# Autodesk Inventor assembly: Rover
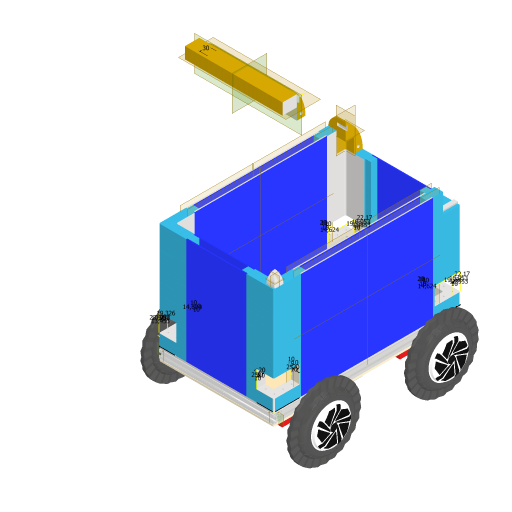
[picture p0: Inventor's stored thumbnail of the model, 512x512]
Saved by Autodesk Inventor 2023.2 (Build 272271030, 271C)
## iProperties
Created: 2024-10-30
Part Number: Rover
Document SubType Name: Assembly
Designer: I9232
Author: I9232
## Documents named in this file (21)
- D:\!Rover\Rover\Rover_construction\Rover.iam
- D:\!Rover\Rover\Rover_construction\platform.ipt
- D:\!Rover\Rover\Rover_construction\Motor, BLDC, Hoverboard Wheel, 8.0in.ipt
- D:\!Rover\Rover\Rover_construction\Profil 20x20.ipt
- D:\!Rover\Rover\Rover_construction\Крепление мотора.iam
- D:\!Rover\Rover\Rover_construction\Copter.ipt
- D:\!Rover\Rover\Rover_construction\Korpus.ipt
- D:\!Rover\Rover\Rover_construction\Уголок для профиля.ipt
- D:\!Rover\Rover\Rover_construction\Профиль 30x30\Профиль 30x30.ipt
- D:\!Rover\Rover\Rover_construction\Т-образный соединитель\Т-образный соединитель.ipt
- D:\!Rover\Rover\Rover_construction\KRAVT_holder_2 (1) (2).ipt
- D:\!Rover\Rover\Rover_construction\столик.ipt
- D:\!Rover\Rover\Rover_construction\Подъёмник.iam
- D:\!Rover\Rover\Rover_construction\Столбик.ipt
- D:\!Rover\Rover\Rover_construction\Боковая часть корпуса.ipt
- D:\!Rover\Rover\Rover_construction\Край задней части корпуса.ipt
- D:\!Rover\Rover\Rover_construction\кубик.ipt
- D:\!Rover\Rover\Rover_construction\Передняя_Задняя фанера.ipt
- D:\!Rover\Rover\Rover_construction\Проставка для боковых фанер.ipt
- D:\!Rover\Rover\Rover_construction\Крышка.ipt
- D:\!Rover\Rover\Rover_construction\Уголок крышки.ipt
## Components (48 placed, 21 different names)
1. platform:1 — Совмещение:1, Совмещение:2, Совмещение:169, Заподлицо:1, Заподлицо:2, Совмещение:170, Совмещение:171, Совмещение:172, Заподлицо:3, Заподлицо:4, Заподлицо:5, Заподлицо:6, Совмещение:180, Заподлицо:11, Совмещение:189, Заподлицо:24, Заподлицо:25, Совмещение:190, Заподлицо:26, Заподлицо:27, Заподлицо:28, Совмещение:191, Заподлицо:29, Совмещение:192, Заподлицо:30, Заподлицо:31, Совмещение:205, Совмещение:206, Заподлицо:33, Заподлицо:34, Заподлицо:37
2. Copter:1 — Совмещение:213, Совмещение:214
3. Корпус:1 — Совмещение:210, Совмещение:211, Заподлицо:33, Заподлицо:34, Совмещение:212
4. Т-образный соединитель:1 — Заподлицо:21, Совмещение:186, Совмещение:188
5. Т-образный соединитель:2 — Заподлицо:22, Совмещение:187, Заподлицо:23
6. KRAVT_holder_2 (1) (2):1 — Совмещение:206, Заподлицо:32, Совмещение:209
7. KRAVT_holder_2 (1) (2):2 — Совмещение:205, Совмещение:207, Совмещение:208
8. столик:1 — Совмещение:210, Совмещение:211, Совмещение:213
9. Copter:2 — Совмещение:214
10. Подъёмник:1 [sub-assembly]
11. platform:2 — Совмещение:221, Заподлицо:37, Заподлицо:38, Совмещение:222, Совмещение:224, Совмещение:226, Совмещение:230, Заподлицо:40, Заподлицо:41, Совмещение:268, Совмещение:306, Заподлицо:50, Заподлицо:51, Совмещение:307, Совмещение:308, Заподлицо:52
12. Столбик:1 — Совмещение:222, Совмещение:226, Заподлицо:41, Совмещение:249, Совмещение:251, Совмещение:262, Совмещение:264, Совмещение:282, Совмещение:283, Совмещение:289, Заподлицо:48, Совмещение:292, Заподлицо:49
13. Столбик:3 — Совмещение:224, Совмещение:230, Заподлицо:40, Совмещение:266, Совмещение:273, Совмещение:275, Совмещение:277, Совмещение:281, Совмещение:294, Совмещение:299, Совмещение:302, Совмещение:305, Совмещение:309, Заподлицо:53
14. Боковая часть корпуса:1 — Совмещение:292, Заподлицо:49
15. Боковая часть корпуса:2 — Совмещение:273, Совмещение:281, Совмещение:293, Совмещение:304
16. Боковая часть корпуса:3 — Совмещение:289, Заподлицо:48, Совмещение:296
17. Боковая часть корпуса:4 — Совмещение:275, Совмещение:277
18. Край задней части корпуса:1 — Совмещение:249, Совмещение:304, Совмещение:305
19. кубик:1 — Совмещение:251
20. Передняя_Задняя фанера:1 — Совмещение:264
21. Передняя_Задняя фанера:2 — Совмещение:262, Совмещение:282, Совмещение:283
22. Передняя_Задняя фанера:4 — Совмещение:266, Совмещение:268
23. Проставка для боковых фанер:1 — Совмещение:293, Совмещение:294
24. Проставка для боковых фанер:2 — Совмещение:296
25. Крышка:1 — Совмещение:299, Совмещение:310
26. Уголок крышки:1 — Совмещение:302, Совмещение:309, Заподлицо:53
27. Столбик:4 — Совмещение:306, Заподлицо:50, Заподлицо:51
28. Столбик:5 — Совмещение:307, Совмещение:308, Заподлицо:52, Совмещение:310
29. Мотор гироскутера — Совмещение:196, Совмещение:197, Совмещение:198
30. Motor, BLDC, Hoverboard Wheel, 8.0in:4 — Совмещение:199, Совмещение:200, Совмещение:201
31. Motor, BLDC, Hoverboard Wheel, 8.0in:5 — Совмещение:193, Совмещение:194, Совмещение:195
32. Motor, BLDC, Hoverboard Wheel, 8.0in:6 — Совмещение:202, Совмещение:203, Совмещение:204
33. Profil 20x20:1 — Симметрия:3, Заподлицо:14, Совмещение:184, Заподлицо:18
34. Profil 20x20:2 — Симметрия:3, Заподлицо:12, Совмещение:181, Заподлицо:13
35. Profil 20x20:3 — Заподлицо:18
36. Профиль 30x30:5 — Совмещение:179, Совмещение:180, Заподлицо:11, Заподлицо:21, Заподлицо:23
37. Профиль 30x30:2 — Совмещение:171, Совмещение:173, Заподлицо:3, Заподлицо:7, Заподлицо:12, Совмещение:181, Совмещение:209, Заподлицо:35, Заподлицо:38
38. Профиль 30x30:3 — Совмещение:170, Заподлицо:5, Заподлицо:6, Совмещение:175, Совмещение:186, Совмещение:188, Совмещение:212, Совмещение:218
39. Профиль 30x30:4 — Совмещение:172, Совмещение:174, Заподлицо:4, Совмещение:178, Заподлицо:13, Заподлицо:14, Совмещение:184, Совмещение:208, Совмещение:217, Совмещение:219
40. Профиль 30x30:1 — Совмещение:169, Заподлицо:1, Заподлицо:2, Совмещение:173, Совмещение:174, Заподлицо:8, Совмещение:179, Заподлицо:22, Совмещение:187, Совмещение:216, Совмещение:220, Заподлицо:36
41. Крепление мотора:1 [sub-assembly] — Совмещение:189, Заподлицо:24, Заподлицо:25, Совмещение:199, Совмещение:200, Совмещение:201
42. Крепление мотора:2 [sub-assembly] — Совмещение:190, Заподлицо:26, Заподлицо:27, Совмещение:196, Совмещение:197, Совмещение:198
43. Крепление мотора:3 [sub-assembly] — Заподлицо:28, Совмещение:191, Заподлицо:29, Совмещение:202, Совмещение:203, Совмещение:204
44. Крепление мотора:4 [sub-assembly] — Совмещение:192, Заподлицо:30, Заподлицо:31, Совмещение:193, Совмещение:194, Совмещение:195
45. Уголок для профиля:1 — Заподлицо:8, Совмещение:178, Совмещение:216, Совмещение:221
46. Уголок для профиля:2 — Совмещение:175, Заподлицо:7
47. Уголок для профиля:3 — Совмещение:220, Заподлицо:35, Заподлицо:36
48. Уголок для профиля:4 — Совмещение:217, Совмещение:218, Совмещение:219
## Relationships (119: Mate 79, Flush 39, Symmetry 1)
- Совмещение:1 [Mate]: platform:1
- Совмещение:2 [Mate]: platform:1
- Симметрия:3 [Symmetry]: Profil 20x20:1 ↔ Profil 20x20:2
- Совмещение:169 [Mate]: platform:1 ↔ Профиль 30x30:1
- Заподлицо:1 [Flush]: platform:1 ↔ Профиль 30x30:1
- Заподлицо:2 [Flush]: platform:1 ↔ Профиль 30x30:1
- Совмещение:170 [Mate]: platform:1 ↔ Профиль 30x30:3
- Совмещение:171 [Mate]: platform:1 ↔ Профиль 30x30:2
- Совмещение:172 [Mate]: platform:1 ↔ Профиль 30x30:4
- Совмещение:173 [Mate]: Профиль 30x30:2 ↔ Профиль 30x30:1
- Заподлицо:3 [Flush]: platform:1 ↔ Профиль 30x30:2
- Совмещение:174 [Mate]: Профиль 30x30:4 ↔ Профиль 30x30:1
- Заподлицо:4 [Flush]: platform:1 ↔ Профиль 30x30:4
- Заподлицо:5 [Flush]: platform:1 ↔ Профиль 30x30:3
- Заподлицо:6 [Flush]: platform:1 ↔ Профиль 30x30:3
- Совмещение:175 [Mate]: Профиль 30x30:3 ↔ Уголок для профиля:2
- Заподлицо:7 [Flush]: Профиль 30x30:2 ↔ Уголок для профиля:2
- Заподлицо:8 [Flush]: Профиль 30x30:1 ↔ Уголок для профиля:1
- Совмещение:178 [Mate]: Профиль 30x30:4 ↔ Уголок для профиля:1
- Совмещение:179 [Mate]: Профиль 30x30:5 ↔ Профиль 30x30:1
- Совмещение:180 [Mate]: platform:1 ↔ Профиль 30x30:5
- Заподлицо:11 [Flush]: platform:1 ↔ Профиль 30x30:5
- Заподлицо:12 [Flush]: Profil 20x20:2 ↔ Профиль 30x30:2
- Совмещение:181 [Mate]: Profil 20x20:2 ↔ Профиль 30x30:2
- Заподлицо:13 [Flush]: Profil 20x20:2 ↔ Профиль 30x30:4
- Заподлицо:14 [Flush]: Profil 20x20:1 ↔ Профиль 30x30:4
- Совмещение:184 [Mate]: Profil 20x20:1 ↔ Профиль 30x30:4
- Заподлицо:18 [Flush] (-200 mm): Profil 20x20:1 ↔ Profil 20x20:3
- Заподлицо:21 [Flush]: Т-образный соединитель:1 ↔ Профиль 30x30:5
- Совмещение:186 [Mate]: Т-образный соединитель:1 ↔ Профиль 30x30:3
- Заподлицо:22 [Flush]: Т-образный соединитель:2 ↔ Профиль 30x30:1
- Совмещение:187 [Mate]: Т-образный соединитель:2 ↔ Профиль 30x30:1
- Заподлицо:23 [Flush]: Т-образный соединитель:2 ↔ Профиль 30x30:5
- Совмещение:188 [Mate]: Т-образный соединитель:1 ↔ Профиль 30x30:3
- Совмещение:189 [Mate]: platform:1 ↔ Крепление мотора:1
- Заподлицо:24 [Flush] (30 mm): platform:1 ↔ Крепление мотора:1
- Заподлицо:25 [Flush]: platform:1 ↔ Крепление мотора:1
- Совмещение:190 [Mate]: platform:1 ↔ Крепление мотора:2
- Заподлицо:26 [Flush] (30 mm): platform:1 ↔ Крепление мотора:2
- Заподлицо:27 [Flush]: platform:1 ↔ Крепление мотора:2
- Заподлицо:28 [Flush] (30 mm): platform:1 ↔ Крепление мотора:3
- Совмещение:191 [Mate]: platform:1 ↔ Крепление мотора:3
- Заподлицо:29 [Flush]: platform:1 ↔ Крепление мотора:3
- Совмещение:192 [Mate]: platform:1 ↔ Крепление мотора:4
- Заподлицо:30 [Flush]: platform:1 ↔ Крепление мотора:4
- Заподлицо:31 [Flush] (30 mm): platform:1 ↔ Крепление мотора:4
- Совмещение:193 [Mate]: Motor, BLDC, Hoverboard Wheel, 8.0in:5 ↔ Крепление мотора:4
- Совмещение:194 [Mate]: Motor, BLDC, Hoverboard Wheel, 8.0in:5 ↔ Крепление мотора:4
- Совмещение:195 [Mate]: Motor, BLDC, Hoverboard Wheel, 8.0in:5 ↔ Крепление мотора:4
- Совмещение:196 [Mate]: Мотор гироскутера ↔ Крепление мотора:2
- Совмещение:197 [Mate]: Мотор гироскутера ↔ Крепление мотора:2
- Совмещение:198 [Mate]: Мотор гироскутера ↔ Крепление мотора:2
- Совмещение:199 [Mate]: Motor, BLDC, Hoverboard Wheel, 8.0in:4 ↔ Крепление мотора:1
- Совмещение:200 [Mate]: Motor, BLDC, Hoverboard Wheel, 8.0in:4 ↔ Крепление мотора:1
- Совмещение:201 [Mate]: Motor, BLDC, Hoverboard Wheel, 8.0in:4 ↔ Крепление мотора:1
- Совмещение:202 [Mate]: Motor, BLDC, Hoverboard Wheel, 8.0in:6 ↔ Крепление мотора:3
- Совмещение:203 [Mate]: Motor, BLDC, Hoverboard Wheel, 8.0in:6 ↔ Крепление мотора:3
- Совмещение:204 [Mate]: Motor, BLDC, Hoverboard Wheel, 8.0in:6 ↔ Крепление мотора:3
- Совмещение:205 [Mate]: platform:1 ↔ KRAVT_holder_2 (1) (2):2
- Совмещение:206 [Mate]: platform:1 ↔ KRAVT_holder_2 (1) (2):1
- Заподлицо:32 [Flush]: KRAVT_holder_2 (1) (2):1
- Совмещение:207 [Mate]: KRAVT_holder_2 (1) (2):2
- Совмещение:208 [Mate]: KRAVT_holder_2 (1) (2):2 ↔ Профиль 30x30:4
- Совмещение:209 [Mate]: KRAVT_holder_2 (1) (2):1 ↔ Профиль 30x30:2
- Совмещение:210 [Mate]: Корпус:1 ↔ столик:1
- Совмещение:211 [Mate]: Корпус:1 ↔ столик:1
- Заподлицо:33 [Flush]: platform:1 ↔ Корпус:1
- Заподлицо:34 [Flush]: platform:1 ↔ Корпус:1
- Совмещение:212 [Mate]: Корпус:1 ↔ Профиль 30x30:3
- Совмещение:213 [Mate]: Copter:1 ↔ столик:1
- Совмещение:214 [Mate]: Copter:1 ↔ Copter:2
- Совмещение:216 [Mate]: Профиль 30x30:1 ↔ Уголок для профиля:1
- Совмещение:217 [Mate]: Профиль 30x30:4 ↔ Уголок для профиля:4
- Совмещение:218 [Mate]: Профиль 30x30:3 ↔ Уголок для профиля:4
- Совмещение:219 [Mate]: Профиль 30x30:4 ↔ Уголок для профиля:4
- Совмещение:220 [Mate]: Профиль 30x30:1 ↔ Уголок для профиля:3
- Заподлицо:35 [Flush]: Профиль 30x30:2 ↔ Уголок для профиля:3
- Заподлицо:36 [Flush]: Профиль 30x30:1 ↔ Уголок для профиля:3
- Совмещение:221 [Mate]: platform:2 ↔ Уголок для профиля:1
- Заподлицо:37 [Flush]: platform:1 ↔ platform:2
- Заподлицо:38 [Flush]: platform:2 ↔ Профиль 30x30:2
- Совмещение:222 [Mate]: platform:2 ↔ Столбик:1
- Совмещение:224 [Mate]: platform:2 ↔ Столбик:3
- Совмещение:226 [Mate]: platform:2 ↔ Столбик:1
- Совмещение:230 [Mate]: platform:2 ↔ Столбик:3
- Заподлицо:40 [Flush]: platform:2 ↔ Столбик:3
- Заподлицо:41 [Flush]: platform:2 ↔ Столбик:1
- Совмещение:249 [Mate]: Столбик:1 ↔ Край задней части корпуса:1
- Совмещение:251 [Mate]: Столбик:1 ↔ кубик:1
- Совмещение:262 [Mate]: Столбик:1 ↔ Передняя_Задняя фанера:2
- Совмещение:264 [Mate]: Столбик:1 ↔ Передняя_Задняя фанера:1
- Совмещение:266 [Mate]: Столбик:3 ↔ Передняя_Задняя фанера:4
- Совмещение:268 [Mate]: platform:2 ↔ Передняя_Задняя фанера:4
- Совмещение:273 [Mate]: Столбик:3 ↔ Боковая часть корпуса:2
- Совмещение:275 [Mate]: Столбик:3 ↔ Боковая часть корпуса:4
- Совмещение:277 [Mate]: Столбик:3 ↔ Боковая часть корпуса:4
- Совмещение:281 [Mate]: Столбик:3 ↔ Боковая часть корпуса:2
- Совмещение:282 [Mate]: Столбик:1 ↔ Передняя_Задняя фанера:2
- Совмещение:283 [Mate]: Столбик:1 ↔ Передняя_Задняя фанера:2
- Совмещение:289 [Mate]: Столбик:1 ↔ Боковая часть корпуса:3
- Заподлицо:48 [Flush]: Столбик:1 ↔ Боковая часть корпуса:3
- Совмещение:292 [Mate]: Столбик:1 ↔ Боковая часть корпуса:1
- Заподлицо:49 [Flush]: Столбик:1 ↔ Боковая часть корпуса:1
- Совмещение:293 [Mate]: Боковая часть корпуса:2 ↔ Проставка для боковых фанер:1
- Совмещение:294 [Mate]: Столбик:3 ↔ Проставка для боковых фанер:1
- Совмещение:296 [Mate]: Боковая часть корпуса:3 ↔ Проставка для боковых фанер:2
- Совмещение:299 [Mate]: Столбик:3 ↔ Крышка:1
- Совмещение:302 [Mate]: Столбик:3 ↔ Уголок крышки:1
- Совмещение:304 [Mate]: Боковая часть корпуса:2 ↔ Край задней части корпуса:1
- Совмещение:305 [Mate]: Столбик:3 ↔ Край задней части корпуса:1
- Совмещение:306 [Mate]: platform:2 ↔ Столбик:4
- Заподлицо:50 [Flush]: platform:2 ↔ Столбик:4
- Заподлицо:51 [Flush]: platform:2 ↔ Столбик:4
- Совмещение:307 [Mate]: platform:2 ↔ Столбик:5
- Совмещение:308 [Mate]: platform:2 ↔ Столбик:5
- Заподлицо:52 [Flush]: platform:2 ↔ Столбик:5
- Совмещение:309 [Mate]: Столбик:3 ↔ Уголок крышки:1
- Заподлицо:53 [Flush]: Столбик:3 ↔ Уголок крышки:1
- Совмещение:310 [Mate]: Крышка:1 ↔ Столбик:5
